# Autodesk Inventor assembly: tau2
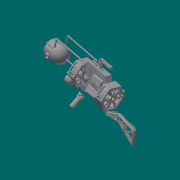
[picture p0: Inventor's stored thumbnail of the model, 180x180]
Saved by Autodesk Inventor 2020.4 (Build 244396010, 396A)
## iProperties
Created: 2022-09-08
Part Number: tau2
Document SubType Name: Assembly
Designer: Val
Author: Val
## Documents named in this file (25)
- C:\Users\Val\Desktop\tau\Tau.iam
- C:\Users\Val\Desktop\tau\external\TopHandle.ipt
- C:\Users\Val\Desktop\tau\Body.ipt
- C:\Users\Val\Desktop\tau\external\FlowMeter.ipt
- C:\Users\Val\Desktop\tau\external\SideHandle.ipt
- C:\Users\Val\Desktop\tau\external\SideHandleBase.ipt
- C:\Users\Val\Desktop\tau\HexCoil.ipt
- C:\Users\Val\Desktop\tau\CoilCover.ipt
- C:\Users\Val\Desktop\tau\Stock.ipt
- C:\Users\Val\Desktop\tau\Stock_MIR.ipt
- C:\Users\Val\Desktop\tau\HoseConnector.ipt
- C:\Users\Val\Desktop\tau\BatteryCover.ipt
- C:\Users\Val\Desktop\tau\BatteryCoverLid.ipt
- C:\Users\Val\Desktop\tau\muzzle.ipt
- C:\Users\Val\Desktop\tau\MuzzleEndBall.ipt
- C:\Users\Val\Desktop\tau\MuzzleEndTube.ipt
- C:\Users\Val\Desktop\tau\ToroidalCore.ipt
- C:\Users\Val\Desktop\tau\MuzzleWireProtector.ipt
- C:\Users\Val\Desktop\tau\TopPipe.ipt
- C:\Users\Val\Desktop\tau\TopPipe_MIR.ipt
- C:\Users\Val\Desktop\tau\external\CO2Cartridge16g.ipt
- C:\Users\Val\Desktop\tau\external\Picatinny2Hole.ipt
- C:\Users\Val\Desktop\tau\BatteryHeatsink.ipt
- C:\Users\Val\Desktop\tau\StockMountPlate.ipt
- C:\Users\Val\Desktop\tau\BodyMirror.ipt
## Components (38 placed, 24 different names)
1. TopHandle:1
2. Body:1 — Mate:1, Mate:3, Mate:4, Mate:6, Mate:15, Mate:26, Mate:30, Flush:35, Mate:37, Mate:38, Mate:47, Mate:55, Angle:4, Mate:56, Mate:57, Mate:79, Mate:80, Mate:81, Mate:82, Mate:83, Mate:84
3. FlowMeter:1 — Mate:3, Mate:4, Mate:6
4. SideHandle:1 — Mate:52, Mate:53
5. HexCoil:1 — Mate:13, Mate:15, Flush:6, Flush:7, Mate:27, Flush:10, Flush:11, Mate:31, Flush:12, Flush:13, Flush:37, Angle:1, Angle:2, Flush:48
6. HexCoil:2 — Flush:6, Flush:7, Mate:22, Flush:8, Mate:24, Flush:9, Mate:25, Flush:35, Mate:72, Mate:73, Mate:74
7. CoilCover:1 — Mate:22, Flush:8, Mate:25, Mate:45
8. CoilCover:2 — Mate:24, Flush:9, Mate:26
9. CoilCover:3 — Mate:31, Flush:12, Flush:13, Flush:36, Mate:33
10. CoilCover:4 — Mate:27, Flush:10, Flush:11, Mate:30, Mate:59
11. Stock:1 — Flush:34, Mate:75, Mate:76
12. Stock_MIR:1 — Mate:60, Mate:61, Mate:77, Mate:78
13. HoseConnector:1 — Flush:36, Mate:33, Flush:37
14. BatteryCover:1 — Flush:38, Flush:39, Flush:44, Flush:45, Mate:66, Mate:67, Mate:68
15. BatteryCover:2 — Flush:38, Mate:35, Flush:40, Flush:41, Mate:64, Mate:65, Angle:6
16. BatteryCover:3 — Flush:39, Mate:36, Flush:42, Flush:43, Mate:39, Flush:46, Flush:47, Mate:69, Mate:70, Mate:71
17. BatteryCoverLid:1 — Mate:35, Flush:40, Flush:41, Mate:36, Flush:42, Flush:43, Flush:44, Flush:45, Mate:37, Mate:38
18. BatteryCoverLid:2 — Mate:39, Flush:46, Flush:47
19. muzzle:1 — Mate:42, Mate:46
20. MuzzleEndBall:1 — Mate:43, Mate:44, Mate:48
21. MuzzleEndTube:1 — Mate:42, Mate:43, Angle:1, Angle:2, Mate:44, Mate:48
22. ToroidalCore:1 — Mate:46
23. ToroidalCore:2 — Mate:45
24. MuzzleWireProtector:1
25. TopPipe:1 — Mate:47
26. TopPipe_MIR:1
27. CO2Cartridge16g:1 — Flush:48
28. Picatinny2Hole:2 — Mate:55, Angle:4, Mate:56
29. Picatinny2Hole:3 — Mate:57, Mate:58, Mate:59
30. Picatinny2Hole:4 — Mate:60, Mate:62
31. Picatinny2Hole:5 — Mate:61, Mate:63
32. SideHandleBase:1 — Mate:52, Mate:53
33. BatteryHeatsink:1 — Mate:64, Mate:65, Angle:6
34. BatteryHeatsink:2 — Mate:66, Mate:67, Mate:68
35. BatteryHeatsink:3 — Mate:69, Mate:70, Mate:71
36. StockMountPlate:1 — Mate:72, Mate:73, Mate:74, Mate:75, Mate:76, Mate:77, Mate:78
37. BodyMirror:1 — Mate:79, Mate:80, Mate:81
38. Picatinny2Hole:6 — Mate:82, Mate:83, Mate:84
## Relationships (86: Mate 58, Flush 23, Angle 4, Symmetry 1)
- Symmetry:1
- Mate:1: Body:1
- Mate:3: Body:1 ↔ FlowMeter:1
- Mate:4: Body:1 ↔ FlowMeter:1
- Mate:6: Body:1 ↔ FlowMeter:1
- Mate:13: HexCoil:1
- Mate:15: Body:1 ↔ HexCoil:1
- Flush:6: HexCoil:1 ↔ HexCoil:2
- Flush:7: HexCoil:1 ↔ HexCoil:2
- Mate:22: HexCoil:2 ↔ CoilCover:1
- Flush:8: HexCoil:2 ↔ CoilCover:1
- Mate:24: HexCoil:2 ↔ CoilCover:2
- Flush:9: HexCoil:2 ↔ CoilCover:2
- Mate:25: HexCoil:2 ↔ CoilCover:1
- Mate:26: Body:1 ↔ CoilCover:2
- Mate:27: HexCoil:1 ↔ CoilCover:4
- Flush:10: HexCoil:1 ↔ CoilCover:4
- Flush:11: HexCoil:1 ↔ CoilCover:4
- Mate:30: Body:1 ↔ CoilCover:4
- Mate:31: HexCoil:1 ↔ CoilCover:3
- Flush:12: HexCoil:1 ↔ CoilCover:3
- Flush:13: HexCoil:1 ↔ CoilCover:3
- Flush:34: Stock:1
- Flush:35: Body:1 ↔ HexCoil:2
- Flush:36: CoilCover:3 ↔ HoseConnector:1
- Mate:33: CoilCover:3 ↔ HoseConnector:1
- Flush:37: HexCoil:1 ↔ HoseConnector:1
- Flush:38: BatteryCover:1 ↔ BatteryCover:2
- Flush:39: BatteryCover:1 ↔ BatteryCover:3
- Mate:35: BatteryCover:2 ↔ BatteryCoverLid:1
- Flush:40: BatteryCover:2 ↔ BatteryCoverLid:1
- Flush:41: BatteryCover:2 ↔ BatteryCoverLid:1
- Mate:36: BatteryCover:3 ↔ BatteryCoverLid:1
- Flush:42: BatteryCover:3 ↔ BatteryCoverLid:1
- Flush:43: BatteryCover:3 ↔ BatteryCoverLid:1
- Flush:44: BatteryCover:1 ↔ BatteryCoverLid:1
- Flush:45: BatteryCover:1 ↔ BatteryCoverLid:1
- Mate:37: Body:1 ↔ BatteryCoverLid:1
- Mate:38: Body:1 ↔ BatteryCoverLid:1
- Mate:39: BatteryCover:3 ↔ BatteryCoverLid:2
- Flush:46: BatteryCover:3 ↔ BatteryCoverLid:2
- Flush:47: BatteryCover:3 ↔ BatteryCoverLid:2
- Mate:42: muzzle:1 ↔ MuzzleEndTube:1
- Mate:43: MuzzleEndBall:1 ↔ MuzzleEndTube:1
- Angle:1 (0 deg): HexCoil:1 ↔ MuzzleEndTube:1
- Angle:2 (0 deg): HexCoil:1 ↔ MuzzleEndTube:1
- Mate:44: MuzzleEndBall:1 ↔ MuzzleEndTube:1
- Mate:45: CoilCover:1 ↔ ToroidalCore:2
- Mate:46: muzzle:1 ↔ ToroidalCore:1
- Mate:47: Body:1 ↔ TopPipe:1
- Mate:48: MuzzleEndBall:1 ↔ MuzzleEndTube:1
- Flush:48: HexCoil:1 ↔ CO2Cartridge16g:1
- Mate:52: SideHandle:1 ↔ SideHandleBase:1
- Mate:53: SideHandle:1 ↔ SideHandleBase:1
- Mate:55: Body:1 ↔ Picatinny2Hole:2
- Angle:4 (0 deg): Body:1 ↔ Picatinny2Hole:2
- Mate:56: Body:1 ↔ Picatinny2Hole:2
- Mate:57: Body:1 ↔ Picatinny2Hole:3
- Mate:58: Picatinny2Hole:3
- Mate:59: CoilCover:4 ↔ Picatinny2Hole:3
- Mate:60: Stock_MIR:1 ↔ Picatinny2Hole:4
- Mate:61: Stock_MIR:1 ↔ Picatinny2Hole:5
- Mate:62: Picatinny2Hole:4
- Mate:63: Picatinny2Hole:5
- Mate:64: BatteryCover:2 ↔ BatteryHeatsink:1
- Mate:65: BatteryCover:2 ↔ BatteryHeatsink:1
- Angle:6 (0 deg): BatteryCover:2 ↔ BatteryHeatsink:1
- Mate:66: BatteryCover:1 ↔ BatteryHeatsink:2
- Mate:67: BatteryCover:1 ↔ BatteryHeatsink:2
- Mate:68: BatteryCover:1 ↔ BatteryHeatsink:2
- Mate:69: BatteryCover:3 ↔ BatteryHeatsink:3
- Mate:70: BatteryCover:3 ↔ BatteryHeatsink:3
- Mate:71: BatteryCover:3 ↔ BatteryHeatsink:3
- Mate:72: HexCoil:2 ↔ StockMountPlate:1
- Mate:73: HexCoil:2 ↔ StockMountPlate:1
- Mate:74: HexCoil:2 ↔ StockMountPlate:1
- Mate:75: Stock:1 ↔ StockMountPlate:1
- Mate:76: Stock:1 ↔ StockMountPlate:1
- Mate:77: Stock_MIR:1 ↔ StockMountPlate:1
- Mate:78: Stock_MIR:1 ↔ StockMountPlate:1
- Mate:79: Body:1 ↔ BodyMirror:1
- Mate:80: Body:1 ↔ BodyMirror:1
- Mate:81: Body:1 ↔ BodyMirror:1
- Mate:82: Body:1 ↔ Picatinny2Hole:6
- Mate:83: Body:1 ↔ Picatinny2Hole:6
- Mate:84: Body:1 ↔ Picatinny2Hole:6
